# Autodesk Inventor assembly: case_assembly
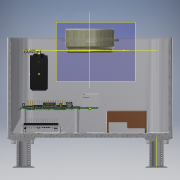
[picture p0: Inventor's stored thumbnail of the model, 180x180]
Saved by Autodesk Inventor 2019 (Build 230136000, 136)
## iProperties
Created: 2019-01-02
Part Number: case_assembly
Document SubType Name: Assembly
Designer: jmc
Author: jmc
## Documents named in this file (14)
- D:\Inventor\Projects\CatFeeder\version2 (fixed enclosure)\version2_newcone.iam
- D:\Inventor\Projects\CatFeeder\Case\version2\case.ipt
- D:\Inventor\Projects\3party\Boards\ArduinoNano\arduino nano.iam
- D:\Inventor\Projects\3party\Boards\Raspberry Pi 3\Raspberry Pi 3.ipt
- D:\Inventor\Projects\3party\Trasformer\Transformer.ipt
- D:\Inventor\Projects\CatFeeder\Case\version2\case_top.ipt
- D:\Inventor\Projects\CatFeeder\Case\version2\case_bottom.ipt
- D:\Inventor\Projects\CatFeeder\Case\version2\Pata.ipt
- D:\Inventor\Projects\CatFeeder\Case\version2\pata_macho.ipt
- D:\Inventor\Projects\CatFeeder\JarCone\version2\cono_nuevo.ipt
- D:\Inventor\Projects\CatFeeder\JarCone\version2\adaptador_cono.ipt
- D:\Inventor\Projects\CatFeeder\Jar\Jar.ipt
- D:\Inventor\Projects\3party\Servos\MG995.ipt
- D:\Inventor\Projects\CatFeeder\Trap\version2\trapdoor_servo.ipt
## Components (19 placed, 13 different names)
1. MG995:1 — Flush:6
2. trapdoor_servo:1 — Flush:6, Flush:8, Flush:9
3. case:1
4. case_top:1 — Rigid:10, Flush:2, Flush:3, Rigid:14, Flush:4, Flush:5
5. cono_nuevo:1 — Rigid:12, Rigid:13
6. adaptador_cono:1 — Rigid:10, Flush:2, Flush:3, Rigid:13, Flush:4, Flush:5, Flush:8
7. Jar:1 — Rigid:12
8. case_bottom:1 — Rigid:1, Rigid:3, Rigid:4, Flush:1, Rotational:1, Rigid:6, Rigid:7, Rigid:8, Rigid:14
9. arduino nano:1 [sub-assembly] — Rigid:4
10. Raspberry Pi 3:1 — Rigid:1
11. Transformer:1 — Rigid:3
12. pata_macho:4 — Rotational:5
13. pata_macho:3 — Rotational:3
14. pata_macho:2 — Rotational:4
15. pata_macho:1 — Rotational:2
16. Pata:1 — Flush:1, Rotational:1, Rotational:2
17. Pata:2 — Rigid:8, Rotational:5
18. Pata:3 — Rigid:7, Rotational:3
19. Pata:4 — Rigid:6, Rotational:4
## Relationships (23: WeldJoint 10, Flush 8, RevoluteJoint 5)
- Rigid:1 [WeldJoint]: case_bottom:1 ↔ Raspberry Pi 3:1
- Rigid:3 [WeldJoint]: case_bottom:1 ↔ Transformer:1
- Rigid:4 [WeldJoint]: case_bottom:1 ↔ arduino nano:1
- Flush:1: case_bottom:1 ↔ Pata:1
- Rotational:1 [RevoluteJoint]: case_bottom:1 ↔ Pata:1
- Rigid:6 [WeldJoint]: case_bottom:1 ↔ Pata:4
- Rigid:7 [WeldJoint]: case_bottom:1 ↔ Pata:3
- Rigid:8 [WeldJoint]: case_bottom:1 ↔ Pata:2
- Rotational:2 [RevoluteJoint]: pata_macho:1 ↔ Pata:1
- Rotational:3 [RevoluteJoint]: pata_macho:3 ↔ Pata:3
- Rotational:4 [RevoluteJoint]: pata_macho:2 ↔ Pata:4
- Rotational:5 [RevoluteJoint]: pata_macho:4 ↔ Pata:2
- Rigid:10 [WeldJoint]: case_top:1 ↔ adaptador_cono:1
- Rigid:12 [WeldJoint]: cono_nuevo:1 ↔ Jar:1
- Flush:2: case_top:1 ↔ adaptador_cono:1
- Flush:3: case_top:1 ↔ adaptador_cono:1
- Rigid:13 [WeldJoint]: cono_nuevo:1 ↔ adaptador_cono:1
- Rigid:14 [WeldJoint]: case_top:1 ↔ case_bottom:1
- Flush:4: case_top:1 ↔ adaptador_cono:1
- Flush:5: case_top:1 ↔ adaptador_cono:1
- Flush:6: MG995:1 ↔ trapdoor_servo:1
- Flush:8: trapdoor_servo:1 ↔ adaptador_cono:1
- Flush:9: trapdoor_servo:1
## Named parameters: HOLE_TOLERANCE = 0.15 mm, CASE_TOLERANCE = 0.08 mm
